# Autodesk Inventor assembly: PivotAssembly
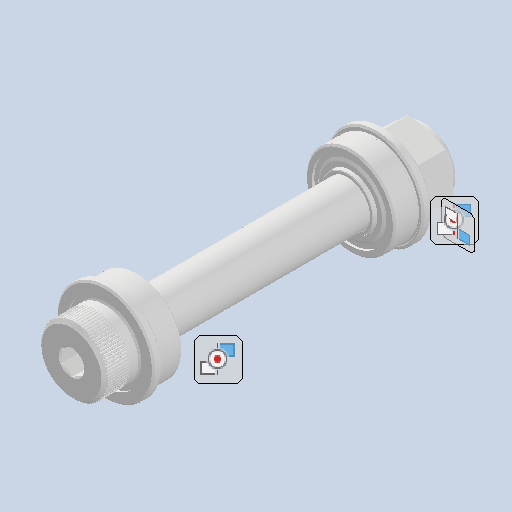
[picture p0: Inventor's stored thumbnail of the model, 512x512]
Saved by Autodesk Inventor 2025.1 (Build 291241020, 241B)
## iProperties
Created: 2023-03-28
Part Number: PivotAssembly
Document SubType Name: Assembly
Designer: Dave
Author: Dave
## Documents named in this file (4)
- C:\Users\t205b\OneDrive\Documents\Github\BehrendURCMechanical\CAD\Chassis V3\CH3-PivotBoltNutWasher.iam
- C:\Users\t205b\OneDrive\Documents\Github\BehrendURCMechanical\CAD\Chassis V3\Pivot Files and Assembly\57155K337_Stainless Steel Ball Bearing1.ipt
- C:\Users\t205b\OneDrive\Documents\Github\BehrendURCMechanical\CAD\Chassis V3\Pivot Files and Assembly\91259A546_Alloy Steel Shoulder Screw1.ipt
- C:\Users\t205b\OneDrive\Documents\Github\BehrendURCMechanical\CAD\Chassis V3\Pivot Files and Assembly\91831A011_18-8 Stainless Steel Nylon-Insert Locknut (1).ipt
## Components (4 placed, 3 different names)
1. 57155K337_Stainless Steel Ball Bearing1:1 — Mate:3, Mate:4
2. 91259A546_Alloy Steel Shoulder Screw1:1 — Mate:1, Mate:3, Mate:13, Mate:15
3. 91831A011_18-8 Stainless Steel Nylon-Insert Locknut (1):1 — Mate:13
4. 57155K337_Stainless Steel Ball Bearing1:2 — Mate:1, Mate:4, Mate:15
## Relationships (5: Mate 5)
- Mate:1: 91259A546_Alloy Steel Shoulder Screw1:1 ↔ 57155K337_Stainless Steel Ball Bearing1:2
- Mate:3: 57155K337_Stainless Steel Ball Bearing1:1 ↔ 91259A546_Alloy Steel Shoulder Screw1:1
- Mate:4 (-39.751 mm): 57155K337_Stainless Steel Ball Bearing1:1 ↔ 57155K337_Stainless Steel Ball Bearing1:2
- Mate:13: 91259A546_Alloy Steel Shoulder Screw1:1 ↔ 91831A011_18-8 Stainless Steel Nylon-Insert Locknut (1):1
- Mate:15: 91259A546_Alloy Steel Shoulder Screw1:1 ↔ 57155K337_Stainless Steel Ball Bearing1:2
